# Autodesk Inventor assembly: Intrepid
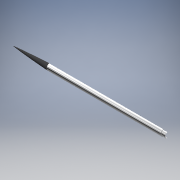
[picture p0: Inventor's stored thumbnail of the model, 180x180]
Saved by Autodesk Inventor 2017 SP1 (Build 210196100, 196)
## iProperties
Created: 2016-10-29
Part Number: Intrepid
Document SubType Name: Assembly
Designer: cflannery
Author: cflannery
## Documents named in this file (6)
- D:\Triton_Rocket_Club\Propulsion\Launches\8-inch-flight\Design\CAD\Vehicle\Intrepid.iam
- D:\Triton_Rocket_Club\Propulsion\Launches\8-inch-flight\Design\CAD\Vehicle\Structures\motor.iam
- D:\Triton_Rocket_Club\Propulsion\Launches\8-inch-flight\Design\CAD\Vehicle\Structures\motor_casing.ipt
- D:\Triton_Rocket_Club\Propulsion\Launches\8-inch-flight\Design\CAD\Vehicle\Structures\recovery_casing.ipt
- D:\Triton_Rocket_Club\Propulsion\Launches\8-inch-flight\Design\CAD\Vehicle\Structures\section_adapter.ipt
- D:\Triton_Rocket_Club\Propulsion\Launches\8-inch-flight\Design\CAD\Vehicle\Structures\nosecone_0.75.ipt
## Components (5 placed, 5 different names)
1. motor:1 [sub-assembly] — Mate:1, Flush:1, Mate:8
2. motor_casing:1 — Mate:1, Flush:1, Mate:2, Mate:3, Mate:4, Mate:8, Mate:9
3. recovery_casing:1 — Mate:2, Mate:6, Mate:10, Mate:11, Mate:12
4. section_adapter:1 — Mate:3, Mate:4, Mate:9, Mate:10, Mate:11
5. nosecone_0.75:1 — Mate:6, Mate:12
## Relationships (11: Mate 10, Flush 1)
- Mate:1: motor:1 ↔ motor_casing:1
- Flush:1: motor:1 ↔ motor_casing:1
- Mate:2: motor_casing:1 ↔ recovery_casing:1
- Mate:3: motor_casing:1 ↔ section_adapter:1
- Mate:4: motor_casing:1 ↔ section_adapter:1
- Mate:6: recovery_casing:1 ↔ nosecone_0.75:1
- Mate:8: motor:1 ↔ motor_casing:1
- Mate:9: motor_casing:1 ↔ section_adapter:1
- Mate:10: recovery_casing:1 ↔ section_adapter:1
- Mate:11: recovery_casing:1 ↔ section_adapter:1
- Mate:12: recovery_casing:1 ↔ nosecone_0.75:1
